# Autodesk Inventor assembly: outer
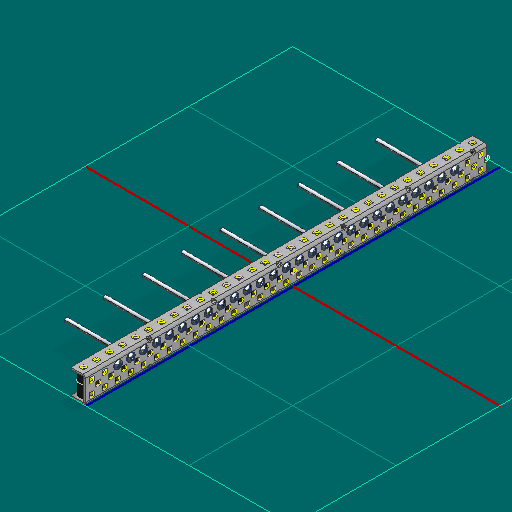
[picture p0: Inventor's stored thumbnail of the model, 512x512]
Saved by Autodesk Inventor 2025 (Build 290162000, 162)
## iProperties
Created: 2024-08-20
Part Number: outer
Document SubType Name: Assembly
Designer: averey
Author: averey
## Documents named in this file (9)
- C:\Users\avere\vex_robotics_high_stakes\hardware\cad\bots\ENIGMA\chassis\drivetrain\drivebay\outer.iam
- C:\Users\avere\vex_robotics_high_stakes\hardware\cad\VEX-CAD-Inventor\Motion\Spacers\Spacer Nylon .375 OD\NSpacer .375 OD x .375.ipt
- C:\Users\avere\vex_robotics_high_stakes\hardware\cad\VEX-CAD-Inventor\Motion\Spacers\Spacer Nylon .375 OD.ipt
- C:\Users\avere\vex_robotics_high_stakes\hardware\cad\VEX-CAD-Inventor\Motion\Spacers\Spacer Nylon .375 OD\NSpacer .375 OD x .500.ipt
- C:\Users\avere\vex_robotics_high_stakes\hardware\cad\VEX-CAD-Inventor\Structure\C Channel\Aluminum 1x2x1\Alu C 1x2x1x31.ipt
- C:\Users\avere\vex_robotics_high_stakes\hardware\cad\_quick_assemblies\bearing_flat_w_hardware.iam
- C:\Users\avere\vex_robotics_high_stakes\hardware\cad\VEX-CAD-Inventor\Structure\Hardware\Screw Steel - Star\SScrew Star Smooth 2.500.ipt
- C:\Users\avere\vex_robotics_high_stakes\hardware\cad\VEX-CAD-Inventor\Structure\Hardware\Screw Steel - Star.ipt
- C:\Users\avere\vex_robotics_high_stakes\hardware\cad\VEX-CAD-Inventor\Structure\Hardware\Nut Thin Nylock.ipt
## Components (32 placed, 6 different names)
1. Alu C 1x2x1x31:1 — Mate:1, Insert:6, Insert:7, Mate:2
2. NSpacer .375 OD x .375:1
3. NSpacer .375 OD x .500:2
4. NSpacer .375 OD x .375:3 — Insert:6
5. NSpacer .375 OD x .500:4
6. Nut Thin Nylock:1 — Insert:9
7. SScrew Star Smooth 2.500:1 — Insert:8
8. bearing_flat_w_hardware:1 [sub-assembly] — Insert:7, Mate:2, Insert:8, Insert:9
9. Nut Thin Nylock:2
10. SScrew Star Smooth 2.500:2
11. bearing_flat_w_hardware:2 [sub-assembly]
12. Nut Thin Nylock:3
13. SScrew Star Smooth 2.500:3
14. bearing_flat_w_hardware:3 [sub-assembly]
15. Nut Thin Nylock:4
16. SScrew Star Smooth 2.500:4
17. bearing_flat_w_hardware:4 [sub-assembly]
18. Nut Thin Nylock:5
19. SScrew Star Smooth 2.500:5
20. bearing_flat_w_hardware:5 [sub-assembly]
21. Nut Thin Nylock:6
22. SScrew Star Smooth 2.500:6
23. bearing_flat_w_hardware:6 [sub-assembly]
24. Nut Thin Nylock:7
25. SScrew Star Smooth 2.500:7
26. bearing_flat_w_hardware:7 [sub-assembly]
27. Nut Thin Nylock:8
28. SScrew Star Smooth 2.500:8
29. bearing_flat_w_hardware:8 [sub-assembly]
30. Nut Thin Nylock:9
31. SScrew Star Smooth 2.500:9
32. bearing_flat_w_hardware:9 [sub-assembly]
## Component patterns: bearings (9 elements)
## Relationships (9: Insert 7, Mate 2)
- [Insert]: NSpacer .375 OD x .375:1 ↔ NSpacer .375 OD x .500:2
- [Insert]: NSpacer .375 OD x .375:3 ↔ NSpacer .375 OD x .500:4
- [Insert]: Alu C 1x2x1x31:1 ↔ NSpacer .375 OD x .375:1
- Mate:1: Alu C 1x2x1x31:1
- Insert:6: Alu C 1x2x1x31:1 ↔ NSpacer .375 OD x .375:3
- Insert:7: Alu C 1x2x1x31:1 ↔ bearing_flat_w_hardware:1
- Mate:2: Alu C 1x2x1x31:1 ↔ bearing_flat_w_hardware:1
- Insert:8 (1.5875 mm): SScrew Star Smooth 2.500:1 ↔ bearing_flat_w_hardware:1
- Insert:9 (1.27 mm): Nut Thin Nylock:1 ↔ bearing_flat_w_hardware:1
## Named parameters: d17_d15 = 0 mm
